# Autodesk Inventor assembly: 100x0y0z_0x0y0z
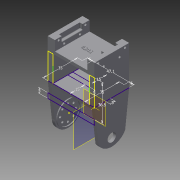
[picture p0: Inventor's stored thumbnail of the model, 180x180]
Saved by Autodesk Inventor 2015 (Build 190159000, 159)
## iProperties
Created: 2016-12-15
Part Number: 100x0y0z_0x0y0z
Document SubType Name: Assembly
Designer: Rudge-Top
Author: Rudge-Top
## Documents named in this file (4)
- C:\Users\Rudge-Top\Documents\RoboticArm\Inventor 2015\Straight Links\100x0y0z_0x0y0z.iam
- C:\Users\Rudge-Top\Documents\RoboticArm\Inventor 2015\Mounts\BaseMount.ipt
- C:\Users\Rudge-Top\Documents\RoboticArm\Inventor 2015\Mounts\Turnmount.ipt
- C:\Users\Rudge-Top\Documents\RoboticArm\Inventor 2015\Straight Links\100x0y0z_0x0y0z.ipt
## Components (3 placed, 3 different names)
1. 100x0y0z_0x0y0z:1 — Mate:1, Flush:1, Flush:2, Mate:2, Flush:3, Flush:4
2. BaseMount:1 — Mate:2, Flush:3, Flush:4
3. Turnmount:1 — Mate:1, Flush:1, Flush:2
## Relationships (6: Flush 4, Mate 2)
- Mate:1: 100x0y0z_0x0y0z:1 ↔ Turnmount:1
- Flush:1: 100x0y0z_0x0y0z:1 ↔ Turnmount:1
- Flush:2: 100x0y0z_0x0y0z:1 ↔ Turnmount:1
- Mate:2: 100x0y0z_0x0y0z:1 ↔ BaseMount:1
- Flush:3: 100x0y0z_0x0y0z:1 ↔ BaseMount:1
- Flush:4: 100x0y0z_0x0y0z:1 ↔ BaseMount:1
